# Autodesk Inventor assembly: A_Airbert
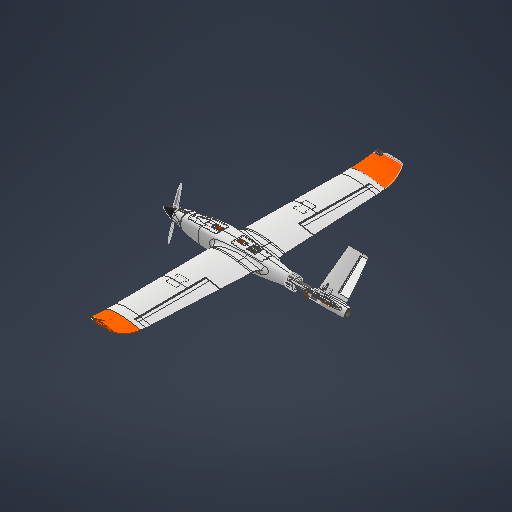
[picture p0: Inventor's stored thumbnail of the model, 512x512]
Saved by Autodesk Inventor 2026 (Build 300175000, 175)
## iProperties
Created: 2025-08-22
Part Number: A_Airbert
Document SubType Name: Assembly
Designer: FAL
Mass: 940.749 g
Surface Area: 6231.37 cm^2
Volume: 1491.38 cm^3
Author: FAL
## Documents named in this file (51)
- C:\Users\FAL\Projekte\Git\AEROLAB\01_AIRCRAFTS\AIR-BERT\CAD\A_Airbert.iam
- C:\Users\FAL\Projekte\Git\AEROLAB\01_AIRCRAFTS\AIR-BERT\CAD\P_Fuselage.ipt
- C:\Users\FAL\Projekte\Git\AEROLAB\01_AIRCRAFTS\AIR-BERT\CAD\P_Carbon_Pipe_Back.ipt
- C:\Users\FAL\Projekte\Git\AEROLAB\01_AIRCRAFTS\AIR-BERT\CAD\extern\P_AP-PR-006_6-2_LH.ipt
- C:\Users\FAL\Projekte\Git\AEROLAB\01_AIRCRAFTS\AIR-BERT\CAD\P_aft_V.ipt
- C:\Users\FAL\Projekte\Git\AEROLAB\01_AIRCRAFTS\AIR-BERT\CAD\extern\P_Akku_Dummy.ipt
- C:\Users\FAL\Projekte\Git\AEROLAB\01_AIRCRAFTS\AIR-BERT\CAD\P_aft_T.ipt
- P_aft_T.ipt
- C:\Users\FAL\Projekte\Git\AEROLAB\01_AIRCRAFTS\AIR-BERT\CAD\extern\P_BLDC_2200KV.ipt
- C:\Users\FAL\Projekte\Git\AEROLAB\01_AIRCRAFTS\AIR-BERT\CAD\extern\P_Receiver_Radiolink.ipt
- C:\Users\FAL\Projekte\Git\AEROLAB\01_AIRCRAFTS\AIR-BERT\CAD\extern\P_ESC_40A.ipt
- C:\Users\FAL\Projekte\Git\AEROLAB\01_AIRCRAFTS\AIR-BERT\CAD\P_aft_X.ipt
- P_aft_X.ipt
- C:\Users\FAL\Projekte\Git\AEROLAB\01_AIRCRAFTS\AIR-BERT\CAD\P_MotorNose.ipt
- C:\Users\FAL\Projekte\Git\AEROLAB\01_AIRCRAFTS\AIR-BERT\CAD\P_Fuselage_cuts.ipt
- P_Fuselage_Cuts.ipt
- C:\Users\FAL\Projekte\Git\AEROLAB\01_AIRCRAFTS\AIR-BERT\CAD\P_Fuselage_Body.ipt
- C:\Users\FAL\Projekte\Git\AEROLAB\01_AIRCRAFTS\AIR-BERT\CAD\P_Fuselage_Nose.ipt
- C:\Users\FAL\Projekte\Git\AEROLAB\01_AIRCRAFTS\AIR-BERT\CAD\extern\P_Servo_SIMPROP.ipt
- C:\Users\FAL\Projekte\Git\AEROLAB\01_AIRCRAFTS\AIR-BERT\CAD\P_Wing_inner.ipt
- C:\Users\FAL\Projekte\Git\AEROLAB\01_AIRCRAFTS\AIR-BERT\CAD\P_Wing_mid.ipt
- C:\Users\FAL\Projekte\Git\AEROLAB\01_AIRCRAFTS\AIR-BERT\CAD\P_Wing_winglet.ipt
- C:\Users\FAL\Projekte\Git\AEROLAB\01_AIRCRAFTS\AIR-BERT\CAD\P_Wing_aileron.ipt
- C:\Users\FAL\Projekte\Git\AEROLAB\01_AIRCRAFTS\AIR-BERT\CAD\P_Fuselage_cap_front.ipt
- C:\Users\FAL\Projekte\Git\AEROLAB\01_AIRCRAFTS\AIR-BERT\CAD\P_Wing_Carbonpipe_A.ipt
- C:\Users\FAL\Projekte\Git\AEROLAB\01_AIRCRAFTS\AIR-BERT\CAD\P_Fuselage_cap_mid.ipt
- C:\Users\FAL\Projekte\Git\AEROLAB\01_AIRCRAFTS\AIR-BERT\CAD\P_Wing_mid_servocap.ipt
- C:\Users\FAL\Projekte\Git\AEROLAB\01_AIRCRAFTS\AIR-BERT\CAD\extern\P_Servo_SIMPROP_lever.ipt
- C:\Users\FAL\Projekte\Git\AEROLAB\01_AIRCRAFTS\AIR-BERT\CAD\P_Wing_mid_servolink.ipt
- C:\Users\FAL\Projekte\Git\AEROLAB\01_AIRCRAFTS\AIR-BERT\CAD\P_Wing_winglet_LEDcap.ipt
- C:\Users\FAL\Projekte\Git\AEROLAB\01_AIRCRAFTS\AIR-BERT\CAD\extern\P_Servo_SIMPROP_27x12.ipt
- C:\Users\FAL\Projekte\Git\AEROLAB\01_AIRCRAFTS\AIR-BERT\CAD\P_Harnes.ipt
- C:\Users\FAL\Projekte\Git\AEROLAB\01_AIRCRAFTS\AIR-BERT\CAD\P_aft_V_rudder.ipt
- C:\Users\FAL\Documents\Inventor\Content Center Files\R2026\de-DE\AS 1420\AS 1420 - 1973 - M3 x 14.ipt
- C:\Users\FAL\Projekte\Git\AEROLAB\01_AIRCRAFTS\AIR-BERT\CAD\P_Wing.ipt
- C:\Users\FAL\Projekte\Git\AEROLAB\01_AIRCRAFTS\AIR-BERT\CAD\extern\P_LED_5.ipt
- C:\Users\FAL\Projekte\Git\AEROLAB\01_AIRCRAFTS\AIR-BERT\CAD\P_Fuselage_body_front.ipt
- C:\Users\FAL\Projekte\Git\AEROLAB\01_AIRCRAFTS\AIR-BERT\CAD\P_fuselage_body_back.ipt
- C:\Users\FAL\Projekte\Git\AEROLAB\01_AIRCRAFTS\AIR-BERT\CAD\P_fuselage_body_mid.ipt
- C:\Users\FAL\Projekte\Git\AEROLAB\01_AIRCRAFTS\AIR-BERT\CAD\openmechanism\A_openmechanism.iam
- C:\Users\FAL\Projekte\Git\AEROLAB\01_AIRCRAFTS\AIR-BERT\CAD\Flightcontroller_PCB\A_Flightcontroller_PCB.iam
- C:\Users\FAL\Projekte\Git\AEROLAB\01_AIRCRAFTS\AIR-BERT\CAD\P_Fuselage_Akkuholder.ipt
- C:\Users\FAL\Projekte\Git\AEROLAB\01_AIRCRAFTS\AIR-BERT\CAD\P_Fuselage_body_pipe_connector_inlet.ipt
- C:\Users\FAL\Projekte\Git\AEROLAB\01_AIRCRAFTS\AIR-BERT\CAD\P_Fuselage_body_pipe_connector_nut.ipt
- C:\Users\FAL\Projekte\Git\AEROLAB\01_AIRCRAFTS\AIR-BERT\CAD\P_Wing_winglet_MIR1.ipt
- C:\Users\FAL\Projekte\Git\AEROLAB\01_AIRCRAFTS\AIR-BERT\CAD\P_Wing_mid_MIR.ipt
- C:\Users\FAL\Projekte\Git\AEROLAB\01_AIRCRAFTS\AIR-BERT\CAD\P_Wing_aileron_MIR.ipt
- C:\Users\FAL\Projekte\Git\AEROLAB\01_AIRCRAFTS\AIR-BERT\CAD\P_Wing_inner_MIR1.ipt
- C:\Users\FAL\Projekte\Git\AEROLAB\01_AIRCRAFTS\AIR-BERT\CAD\P_Wing_winglet_LEDcap_MIR.ipt
- C:\Users\FAL\Projekte\Git\AEROLAB\01_AIRCRAFTS\AIR-BERT\CAD\P_aft_V_rudder_MIR.ipt
- C:\Users\FAL\Projekte\Git\AEROLAB\01_AIRCRAFTS\AIR-BERT\CAD\P_Wing_mid_servocap_MIR.ipt
## Components (53 placed, 47 different names)
1. P_Fuselage_Body:1 — Fluchtend:28, Fluchtend:29, Fluchtend:30, Passend:31, Passend:66
2. P_Fuselage_Cuts:1 — Fluchtend:14, Fluchtend:15, Fluchtend:16
3. P_Fuselage:2 — Fluchtend:11, Fluchtend:12, Fluchtend:13, Passend:15
4. P_Wing:1 — Fluchtend:89, Fluchtend:90, Fluchtend:91
5. A_Flightcontroller_PCB:1 [sub-assembly] — Passend:149, Passend:154
6. P_LED_5:1 — Passend:96
7. P_Akku_Dummy:1 — Passend:147
8. P_ESC_40A:1
9. P_Receiver_Radiolink:1 — Passend:152
10. P_BLDC_2200KV:1 — Passend:12, Passend:31, Fluchtend:83
11. P_Servo_SIMPROP:3 — Passend:139, Passend:141, Passend:142, Passend:143, Passend:145
12. P_Servo_SIMPROP_lever:1 — Passend:137, Passend:138, Passend:142, Passend:143
13. P_Servo_SIMPROP_27x12:1 — Passend:89, Passend:90, Passend:91, Passend:94, Passend:95
14. P_Servo_SIMPROP_27x12:2 — Passend:86, Passend:87, Passend:88, Passend:92, Passend:93
15. P_Servo_SIMPROP_lever:4 — Passend:94, Passend:95
16. P_Servo_SIMPROP_lever:5 — Passend:92, Passend:93
17. P_aft_V_rudder:2 — Passend:64, Passend:65
18. P_Carbon_Pipe_Back:1 — Passend:6, Passend:10, Fluchtend:10, Passend:15, Passend:21, Passend:28, Passend:66, Fluchtend:106
19. P_aft_V:1 — Passend:6, Fluchtend:8, Passend:64, Passend:65, Passend:86, Passend:87, Passend:88, Passend:89, Passend:90, Passend:91, Fluchtend:106
20. P_aft_T:1 — Passend:9, Passend:10, Fluchtend:10
21. P_aft_X:1 — Passend:18, Passend:21, Passend:28
22. P_Fuselage_body_pipe_connector_nut:1 — Fluchtend:120, Fluchtend:121, Fluchtend:122
23. P_Fuselage_body_pipe_connector_inlet:1 — Fluchtend:116, Fluchtend:117, Fluchtend:118, Fluchtend:119
24. P_Fuselage_Akkuholder:1 — Fluchtend:114, Fluchtend:115
25. A_openmechanism:1 [sub-assembly] — Fluchtend:104, Passend:157, Fluchtend:124
26. A_openmechanism:2 [sub-assembly] — Passend:158, Fluchtend:125, Passend:159
27. P_Fuselage_cap_front:1 — Fluchtend:53, Fluchtend:54, Fluchtend:55, Passend:157, Fluchtend:124
28. P_Fuselage_cap_mid:1 — Fluchtend:58, Fluchtend:59, Fluchtend:60, Fluchtend:125, Passend:159
29. P_Fuselage_Nose:1 — Fluchtend:32, Fluchtend:42, Fluchtend:43, Einfügen:1, Einfügen:2
30. P_Fuselage_body_front:1 — Fluchtend:95, Fluchtend:96, Fluchtend:97, Passend:147
31. P_fuselage_body_back:1 — Fluchtend:92, Fluchtend:93, Fluchtend:94, Passend:154
32. P_fuselage_body_mid:1 — Fluchtend:98, Fluchtend:99, Fluchtend:100, Passend:129, Passend:144
33. P_Wing_mid_servocap:1 — Fluchtend:64, Fluchtend:65, Fluchtend:66
34. P_Wing_winglet:1 — Fluchtend:39, Fluchtend:40, Fluchtend:41
35. P_Wing_mid:1 — Fluchtend:36, Fluchtend:37, Fluchtend:38, Passend:134
36. P_Wing_aileron:1 — Fluchtend:44, Fluchtend:45, Fluchtend:46, Passend:133, Passend:134
37. P_Wing_mid_servolink:1 — Passend:137, Passend:138
38. P_Wing_inner:1 — Fluchtend:33, Fluchtend:34, Fluchtend:35, Passend:133, Passend:139, Passend:141, Passend:145
39. P_Wing_Carbonpipe_A:1 — Fluchtend:56, Passend:129, Passend:161
40. P_Wing_Carbonpipe_A:2 — Fluchtend:57, Passend:144, Passend:160
41. P_Wing_winglet_LEDcap:1 — Fluchtend:67, Fluchtend:68, Fluchtend:69, Passend:96
42. P_Harnes:1 — Fluchtend:70, Fluchtend:71, Fluchtend:72
43. P_MotorNose:1 — Passend:22
44. P_AP-PR-006_6-2_LH:1 — Passend:14
45. AS 1420 - Metrisch M3 x 14:1 — Einfügen:1
46. AS 1420 - Metrisch M3 x 14:2 — Einfügen:2
47. P_Wing_mid_servocap_MIR:1 — Passend:156
48. P_Wing_winglet_MIR1:1
49. P_Wing_mid_MIR:1
50. P_Wing_aileron_MIR:1
51. P_Wing_inner_MIR1:1 — Passend:160, Passend:161
52. P_Wing_winglet_LEDcap_MIR:1
53. P_aft_V_rudder_MIR:1
## Relationships (117: Flush 69, Mate 46, Insert 2)
- Passend:6 [Mate]: P_Carbon_Pipe_Back:1 ↔ P_aft_V:1
- Fluchtend:8 [Flush]: P_aft_V:1
- Passend:9 [Mate]: P_aft_T:1
- Passend:10 [Mate]: P_Carbon_Pipe_Back:1 ↔ P_aft_T:1
- Fluchtend:10 [Flush]: P_Carbon_Pipe_Back:1 ↔ P_aft_T:1
- Passend:12 [Mate]: P_BLDC_2200KV:1
- Passend:14 [Mate]: P_AP-PR-006_6-2_LH:1
- Fluchtend:11 [Flush]: P_Fuselage:2
- Fluchtend:12 [Flush]: P_Fuselage:2
- Fluchtend:13 [Flush]: P_Fuselage:2
- Passend:15 [Mate]: P_Fuselage:2 ↔ P_Carbon_Pipe_Back:1
- Passend:18 [Mate]: P_aft_X:1
- Passend:21 [Mate]: P_Carbon_Pipe_Back:1 ↔ P_aft_X:1
- Passend:22 [Mate]: P_MotorNose:1
- Fluchtend:14 [Flush]: P_Fuselage_Cuts:1
- Fluchtend:15 [Flush]: P_Fuselage_Cuts:1
- Fluchtend:16 [Flush]: P_Fuselage_Cuts:1
- Fluchtend:28 [Flush]: P_Fuselage_Body:1
- Fluchtend:29 [Flush]: P_Fuselage_Body:1
- Fluchtend:30 [Flush]: P_Fuselage_Body:1
- Fluchtend:32 [Flush]: P_Fuselage_Nose:1
- Fluchtend:42 [Flush]: P_Fuselage_Nose:1
- Fluchtend:43 [Flush]: P_Fuselage_Nose:1
- Passend:28 [Mate]: P_Carbon_Pipe_Back:1 ↔ P_aft_X:1
- Fluchtend:33 [Flush]: P_Wing_inner:1
- Fluchtend:34 [Flush]: P_Wing_inner:1
- Fluchtend:35 [Flush]: P_Wing_inner:1
- Fluchtend:36 [Flush]: P_Wing_mid:1
- Fluchtend:37 [Flush]: P_Wing_mid:1
- Fluchtend:38 [Flush]: P_Wing_mid:1
- Fluchtend:39 [Flush]: P_Wing_winglet:1
- Fluchtend:40 [Flush]: P_Wing_winglet:1
- Fluchtend:41 [Flush]: P_Wing_winglet:1
- Fluchtend:44 [Flush]: P_Wing_aileron:1
- Fluchtend:45 [Flush]: P_Wing_aileron:1
- Fluchtend:46 [Flush]: P_Wing_aileron:1
- Fluchtend:53 [Flush]: P_Fuselage_cap_front:1
- Fluchtend:54 [Flush]: P_Fuselage_cap_front:1
- Fluchtend:55 [Flush]: P_Fuselage_cap_front:1
- Fluchtend:56 [Flush]: P_Wing_Carbonpipe_A:1
- Fluchtend:57 [Flush]: P_Wing_Carbonpipe_A:2
- Passend:31 [Mate]: P_Fuselage_Body:1 ↔ P_BLDC_2200KV:1
- Fluchtend:83 [Flush]: P_BLDC_2200KV:1
- Fluchtend:58 [Flush]: P_Fuselage_cap_mid:1
- Fluchtend:59 [Flush]: P_Fuselage_cap_mid:1
- Fluchtend:60 [Flush]: P_Fuselage_cap_mid:1
- Fluchtend:64 [Flush]: P_Wing_mid_servocap:1
- Fluchtend:65 [Flush]: P_Wing_mid_servocap:1
- Fluchtend:66 [Flush]: P_Wing_mid_servocap:1
- Fluchtend:67 [Flush]: P_Wing_winglet_LEDcap:1
- Fluchtend:68 [Flush]: P_Wing_winglet_LEDcap:1
- Fluchtend:69 [Flush]: P_Wing_winglet_LEDcap:1
- Fluchtend:70 [Flush]: P_Harnes:1
- Fluchtend:71 [Flush]: P_Harnes:1
- Fluchtend:72 [Flush]: P_Harnes:1
- Passend:64 [Mate]: P_aft_V_rudder:2 ↔ P_aft_V:1
- Passend:65 [Mate]: P_aft_V_rudder:2 ↔ P_aft_V:1
- Passend:66 [Mate]: P_Fuselage_Body:1 ↔ P_Carbon_Pipe_Back:1
- Einfügen:1 [Insert]: P_Fuselage_Nose:1 ↔ AS 1420 - Metrisch M3 x 14:1
- Einfügen:2 [Insert]: P_Fuselage_Nose:1 ↔ AS 1420 - Metrisch M3 x 14:2
- Passend:86 [Mate]: P_Servo_SIMPROP_27x12:2 ↔ P_aft_V:1
- Passend:87 [Mate]: P_Servo_SIMPROP_27x12:2 ↔ P_aft_V:1
- Passend:88 [Mate]: P_Servo_SIMPROP_27x12:2 ↔ P_aft_V:1
- Passend:89 [Mate]: P_Servo_SIMPROP_27x12:1 ↔ P_aft_V:1
- Passend:90 [Mate]: P_Servo_SIMPROP_27x12:1 ↔ P_aft_V:1
- Passend:91 [Mate]: P_Servo_SIMPROP_27x12:1 ↔ P_aft_V:1
- Passend:92 [Mate]: P_Servo_SIMPROP_27x12:2 ↔ P_Servo_SIMPROP_lever:5
- Passend:93 [Mate]: P_Servo_SIMPROP_27x12:2 ↔ P_Servo_SIMPROP_lever:5
- Passend:94 [Mate]: P_Servo_SIMPROP_27x12:1 ↔ P_Servo_SIMPROP_lever:4
- Passend:95 [Mate]: P_Servo_SIMPROP_27x12:1 ↔ P_Servo_SIMPROP_lever:4
- Fluchtend:89 [Flush]: P_Wing:1
- Fluchtend:90 [Flush]: P_Wing:1
- Fluchtend:91 [Flush]: P_Wing:1
- Passend:96 [Mate]: P_LED_5:1 ↔ P_Wing_winglet_LEDcap:1
- Fluchtend:92 [Flush]: P_fuselage_body_back:1
- Fluchtend:93 [Flush]: P_fuselage_body_back:1
- Fluchtend:94 [Flush]: P_fuselage_body_back:1
- Fluchtend:95 [Flush]: P_Fuselage_body_front:1
- Fluchtend:96 [Flush]: P_Fuselage_body_front:1
- Fluchtend:97 [Flush]: P_Fuselage_body_front:1
- Fluchtend:98 [Flush]: P_fuselage_body_mid:1
- Fluchtend:99 [Flush]: P_fuselage_body_mid:1
- Fluchtend:100 [Flush]: P_fuselage_body_mid:1
- Fluchtend:104 [Flush]: A_openmechanism:1
- Fluchtend:106 [Flush]: P_Carbon_Pipe_Back:1 ↔ P_aft_V:1
- Passend:129 [Mate]: P_fuselage_body_mid:1 ↔ P_Wing_Carbonpipe_A:1
- Passend:133 [Mate]: P_Wing_aileron:1 ↔ P_Wing_inner:1
- Passend:134 [Mate]: P_Wing_mid:1 ↔ P_Wing_aileron:1
- Passend:137 [Mate]: P_Servo_SIMPROP_lever:1 ↔ P_Wing_mid_servolink:1
- Passend:138 [Mate] (-1 mm): P_Servo_SIMPROP_lever:1 ↔ P_Wing_mid_servolink:1
- Passend:139 [Mate]: P_Servo_SIMPROP:3 ↔ P_Wing_inner:1
- Passend:141 [Mate]: P_Servo_SIMPROP:3 ↔ P_Wing_inner:1
- Passend:142 [Mate]: P_Servo_SIMPROP:3 ↔ P_Servo_SIMPROP_lever:1
- Passend:143 [Mate]: P_Servo_SIMPROP:3 ↔ P_Servo_SIMPROP_lever:1
- Passend:144 [Mate]: P_fuselage_body_mid:1 ↔ P_Wing_Carbonpipe_A:2
- Passend:145 [Mate]: P_Servo_SIMPROP:3 ↔ P_Wing_inner:1
- Passend:147 [Mate]: P_Akku_Dummy:1 ↔ P_Fuselage_body_front:1
- Passend:149 [Mate]: A_Flightcontroller_PCB:1
- Fluchtend:114 [Flush]: P_Fuselage_Akkuholder:1
- Fluchtend:115 [Flush]: P_Fuselage_Akkuholder:1
- Passend:152 [Mate]: P_Receiver_Radiolink:1
- Passend:154 [Mate] (3 mm): A_Flightcontroller_PCB:1 ↔ P_fuselage_body_back:1
- Fluchtend:116 [Flush]: P_Fuselage_body_pipe_connector_inlet:1
- Fluchtend:117 [Flush]: P_Fuselage_body_pipe_connector_inlet:1
- Fluchtend:118 [Flush]: P_Fuselage_body_pipe_connector_inlet:1
- Fluchtend:119 [Flush]: P_Fuselage_body_pipe_connector_inlet:1
- Fluchtend:120 [Flush]: P_Fuselage_body_pipe_connector_nut:1
- Fluchtend:121 [Flush]: P_Fuselage_body_pipe_connector_nut:1
- Fluchtend:122 [Flush]: P_Fuselage_body_pipe_connector_nut:1
- Passend:156 [Mate]: P_Wing_mid_servocap_MIR:1
- Passend:157 [Mate] (0.1 mm): A_openmechanism:1 ↔ P_Fuselage_cap_front:1
- Fluchtend:124 [Flush]: A_openmechanism:1 ↔ P_Fuselage_cap_front:1
- Passend:158 [Mate]: A_openmechanism:2
- Fluchtend:125 [Flush]: A_openmechanism:2 ↔ P_Fuselage_cap_mid:1
- Passend:159 [Mate] (0.1 mm): A_openmechanism:2 ↔ P_Fuselage_cap_mid:1
- Passend:160 [Mate]: P_Wing_Carbonpipe_A:2 ↔ P_Wing_inner_MIR1:1
- Passend:161 [Mate]: P_Wing_Carbonpipe_A:1 ↔ P_Wing_inner_MIR1:1
